# Autodesk Inventor assembly: Assembly1
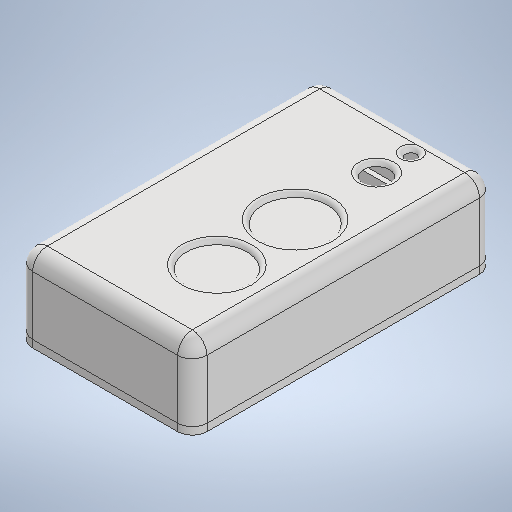
[picture p0: Inventor's stored thumbnail of the model, 512x512]
Saved by Autodesk Inventor 2025.2 (Build 292293000, 293)
## iProperties
Created: 2026-02-22
Part Number: Assembly1
Document SubType Name: Assembly
Designer: naka6
Author: naka6
## Documents named in this file (3)
- C:\Users\naka6\Projects\TimeFaker\Assembly1.iam
- C:\Users\naka6\Projects\TimeFaker\Part1.ipt
- C:\Users\naka6\Projects\TimeFaker\Part2.ipt
## Components (2 placed, 2 different names)
1. Part1:1 — フラッシュ:1
2. Part2:1 — フラッシュ:1
## Relationships (1: Flush 1)
- フラッシュ:1 [Flush]: Part1:1 ↔ Part2:1
